# Autodesk Inventor assembly: Schieber1
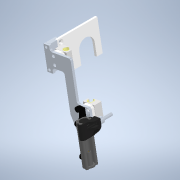
[picture p0: Inventor's stored thumbnail of the model, 180x180]
Saved by Autodesk Inventor 2022 (Build 260153000, 153)
## iProperties
Created: 2022-07-08
Part Number: Schieber1
Document SubType Name: Assembly
Designer: kaebi
Author: kaebi
## Documents named in this file (8)
- C:\Users\kaebi\OneDrive - mci4me.at\03_MCI Master\4.Semester_SS2022\Masterarbeit\Software\CAD_TeachingFactory\Schieber1.iam
- C:\Users\kaebi\OneDrive - mci4me.at\03_MCI Master\4.Semester_SS2022\Masterarbeit\Software\CAD_TeachingFactory\106.016.01_Schienenfuehrung.ipt
- C:\Users\kaebi\OneDrive - mci4me.at\03_MCI Master\4.Semester_SS2022\Masterarbeit\Software\CAD_TeachingFactory\106.019.01_Distanzplatte.ipt
- C:\Users\kaebi\OneDrive - mci4me.at\03_MCI Master\4.Semester_SS2022\Masterarbeit\Software\CAD_TeachingFactory\106.018.01_Schieberelement_oben.ipt
- C:\Users\kaebi\OneDrive - mci4me.at\03_MCI Master\4.Semester_SS2022\Masterarbeit\Software\CAD_TeachingFactory\106.020.01_Winkelaufnahme_Schwert_unten.ipt
- C:\Users\kaebi\OneDrive - mci4me.at\03_MCI Master\4.Semester_SS2022\Masterarbeit\Software\CAD_TeachingFactory\106.030.01_Schwert_oben.ipt
- C:\Users\kaebi\OneDrive - mci4me.at\03_MCI Master\4.Semester_SS2022\Masterarbeit\Software\CAD_TeachingFactory\206.004.02_Kraftlimitierung.iam
- C:\Users\kaebi\OneDrive - mci4me.at\03_MCI Master\4.Semester_SS2022\Masterarbeit\Software\CAD_TeachingFactory\106.035.01_Distanzbolzen_gross.ipt
## Components (9 placed, 7 different names)
1. 106.016.01_Schienenfuehrung:1
2. 106.016.01_Schienenfuehrung:2
3. 106.019.01_Distanzplatte:1 — Passend:23
4. 106.018.01_Schieberelement_oben:1 — Passend:23
5. 106.019.01_Distanzplatte:2
6. 106.020.01_Winkelaufnahme_Schwert_unten:1
7. 106.030.01_Schwert_oben:1
8. 206.004.02_Kraftlimitierung:1 [sub-assembly]
9. 106.035.01_Distanzbolzen_gross:1
## Relationships (23: Mate 23)
- [Mate]: 106.016.01_Schienenfuehrung:1 ↔ 106.019.01_Distanzplatte:1
- [Mate]: 106.016.01_Schienenfuehrung:2 ↔ 106.019.01_Distanzplatte:2
- [Mate]: 106.019.01_Distanzplatte:1 ↔ 106.018.01_Schieberelement_oben:1
- [Mate]: 106.018.01_Schieberelement_oben:1 ↔ 106.020.01_Winkelaufnahme_Schwert_unten:1
- [Mate]: 106.018.01_Schieberelement_oben:1 ↔ 106.020.01_Winkelaufnahme_Schwert_unten:1
- [Mate]: 106.018.01_Schieberelement_oben:1 ↔ 106.020.01_Winkelaufnahme_Schwert_unten:1
- [Mate]: 106.020.01_Winkelaufnahme_Schwert_unten:1 ↔ 106.030.01_Schwert_oben:1
- [Mate]: 106.020.01_Winkelaufnahme_Schwert_unten:1 ↔ 106.030.01_Schwert_oben:1
- [Mate]: 106.020.01_Winkelaufnahme_Schwert_unten:1 ↔ 106.030.01_Schwert_oben:1
- [Mate]: 106.018.01_Schieberelement_oben:1 ↔ 206.004.02_Kraftlimitierung:1
- [Mate]: 206.004.02_Kraftlimitierung:1 ↔ 106.035.01_Distanzbolzen_gross:1
- [Mate]: 206.004.02_Kraftlimitierung:1 ↔ 106.035.01_Distanzbolzen_gross:1
- [Mate]: 106.016.01_Schienenfuehrung:2 ↔ 106.019.01_Distanzplatte:2
- [Mate]: 106.016.01_Schienenfuehrung:2 ↔ 106.019.01_Distanzplatte:2
- [Mate]: 106.016.01_Schienenfuehrung:1 ↔ 106.019.01_Distanzplatte:1
- [Mate]: 106.016.01_Schienenfuehrung:1 ↔ 106.019.01_Distanzplatte:1
- [Mate]: 106.019.01_Distanzplatte:1 ↔ 106.018.01_Schieberelement_oben:1
- [Mate]: 106.016.01_Schienenfuehrung:2 ↔ 106.018.01_Schieberelement_oben:1
- [Mate]: 106.018.01_Schieberelement_oben:1 ↔ 206.004.02_Kraftlimitierung:1
- [Mate]: 106.018.01_Schieberelement_oben:1 ↔ 206.004.02_Kraftlimitierung:1
- [Mate]: 106.018.01_Schieberelement_oben:1 ↔ 106.019.01_Distanzplatte:2
- [Mate]: 106.018.01_Schieberelement_oben:1 ↔ 106.019.01_Distanzplatte:2
- Passend:23 [Mate]: 106.019.01_Distanzplatte:1 ↔ 106.018.01_Schieberelement_oben:1
## Named parameters: d102_d85 = 0 mm, d103_d86 = 0 mm, d110_d111 = 0 mm, d111_d41 = 0 mm, d112_d42 = 0 mm, d113_d43 = 0 mm, d114_d47 = 0 mm, d116_d49 = 0 mm, d117_d55 = 0 mm, d118_d64 = 0 mm, d119_d65 = 0 mm, d120_d19 = 0 mm, d121_d31 = 0 mm, d122_d34 = 0 mm
